# Autodesk Inventor assembly: Assembly1
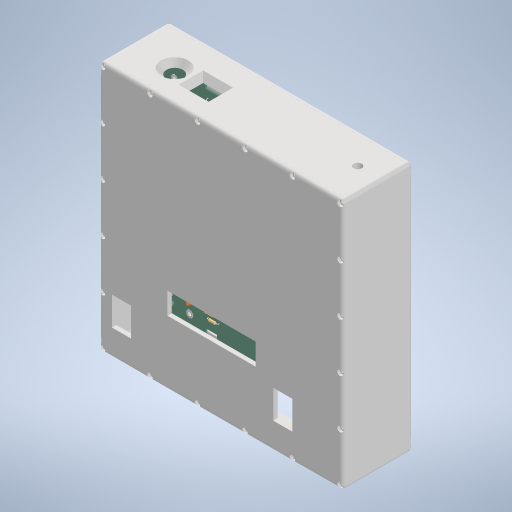
[picture p0: Inventor's stored thumbnail of the model, 512x512]
Saved by Autodesk Inventor 2024 (Build 280153000, 153)
## iProperties
Created: 2023-05-26
Part Number: Assembly1
Document SubType Name: Assembly
Designer: elect
Author: elect
## Documents named in this file (5)
- C:\Users\elect\JDC\Electronics\Projects\righteous_tentacle_colecovision\models\inventor_2024\Assembly1.iam
- C:\Users\elect\JDC\Electronics\Projects\righteous_tentacle_colecovision\models\inventor_2024\base_case\bottom.ipt
- C:\Users\elect\JDC\Electronics\Projects\righteous_tentacle_colecovision\models\inventor_2024\base_case\middle.ipt
- C:\Users\elect\JDC\Electronics\Projects\righteous_tentacle_colecovision\models\inventor_2024\base_case\top.ipt
- C:\Users\elect\JDC\Electronics\Projects\righteous_tentacle_colecovision\models\kicad\coleco_original\coleco_original3.iam
## Components (4 placed, 4 different names)
1. bottom:1 — Mate:2, Mate:3
2. middle:1 — Mate:2, Mate:4, Mate:5, Mate:6
3. coleco_original3:1 [sub-assembly] — Mate:3
4. top:1 — Mate:4, Mate:5, Mate:6
## Relationships (5: Mate 5)
- Mate:2: bottom:1 ↔ middle:1
- Mate:3: bottom:1 ↔ coleco_original3:1
- Mate:4: middle:1 ↔ top:1
- Mate:5: middle:1 ↔ top:1
- Mate:6: middle:1 ↔ top:1
